# Autodesk Inventor assembly: sensory_platform
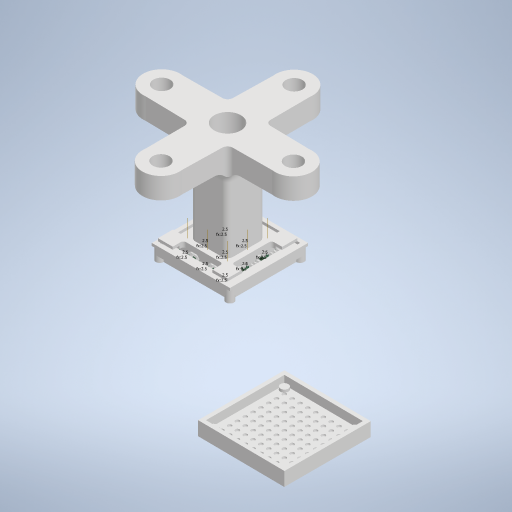
[picture p0: Inventor's stored thumbnail of the model, 512x512]
Saved by Autodesk Inventor 2023.1 (Build 271208000, 208)
## iProperties
Created: 2022-08-08
Part Number: sensory_platform
Document SubType Name: Assembly
Designer: fraaw
Author: fraaw
## Documents named in this file (6)
- C:\Users\swang\OneDrive - Fondazione Istituto Italiano Tecnologia\Desktop\CAD\sensory_platform.iam
- C:\Users\swang\OneDrive - Fondazione Istituto Italiano Tecnologia\Desktop\CAD\franka_mount.ipt
- C:\Users\swang\OneDrive - Fondazione Istituto Italiano Tecnologia\Desktop\CAD\sensor_soldering_mold.ipt
- C:\Users\swang\OneDrive - Fondazione Istituto Italiano Tecnologia\Desktop\CAD\sensor_holder.ipt
- C:\Users\swang\OneDrive - Fondazione Istituto Italiano Tecnologia\Desktop\CAD\sensor_unit.ipt
- C:\Users\swang\OneDrive - Fondazione Istituto Italiano Tecnologia\Desktop\CAD\silicon_mold.ipt
## Components (13 placed, 5 different names)
1. franka_mount:1 — Rigid:1
2. sensor_soldering_mold:1
3. sensor_holder:1 — Rigid:1, Rigid:2
4. silicon_mold:1
5. sensor_unit:1 — Rigid:2
6. sensor_unit:2
7. sensor_unit:3
8. sensor_unit:4
9. sensor_unit:5
10. sensor_unit:6
11. sensor_unit:7
12. sensor_unit:8
13. sensor_unit:9
## Component patterns: (9 elements, first: sensor_unit:1)
## Relationships (2: WeldJoint 2)
- Rigid:1 [WeldJoint] (-5 mm): franka_mount:1 ↔ sensor_holder:1
- Rigid:2 [WeldJoint]: sensor_holder:1 ↔ sensor_unit:1
